# Autodesk Inventor assembly: robot
(part 2 of 2)
- Insert:483: servo frame mg996 centered_MIR_MIR:1 ↔ m2 nuts:23
## Named parameters: d57_d28 = 0 mm, d58_d29 = 0 mm, d59_d16 = 0 mm, d60_d17 = 0 deg, d61_d18 = 0 mm, d62_d19 = 0 mm, d63_d20 = 0 mm, d64_d21 = 0 mm, d65_d22 = 0 mm, d66_d23 = 0 mm, d67_d24 = 0 mm, d68_d25 = 0 mm, d69_d26 = 0 mm, d70_d27 = 0 mm, d71_d5 = 0 mm, d72_d6 = 0 mm, d73_d7 = 0 mm, d74_d8 = 0 mm, d75_d9 = 0 mm, d76_d10 = 0 mm, d77_d11 = 0 mm, d78_d12 = 0 mm, d79_d13 = 0 mm, d80_d14 = 0 mm, d81_d0 = 0 mm, d82_d1 = 0 mm, d83_d2 = 0 mm, d88_d0 = 0 mm, d89_d1 = 0 mm, d90_d2 = 0 mm, d91_d5 = 0 mm, d92_d6 = 0 mm, d93_d7 = 0 mm, d94_d8 = 0 mm, d95_d9 = 0 mm, d96_d10 = 0 mm, d97_d11 = 0 mm, d98_d12 = 0 mm, d99_d13 = 0 mm, d100_d14 = 0 mm, d101_d16 = 0 mm, d102_d17 = 0 deg, d103_d18 = 0 mm, d104_d19 = 0 mm, d105_d20 = 0 mm, d106_d21 = 0 mm, d107_d22 = 0 mm, d108_d23 = 0 mm, d109_d24 = 0 mm, d110_d25 = 0 mm, d111_d26 = 0 mm, d112_d27 = 0 mm, d113_d28 = 0 mm, d114_d29 = 0 mm, d118_d0 = 0 mm, d119_d1 = 0 mm, d120_d2 = 0 mm, d121_d5 = 0 mm, d122_d6 = 0 mm, d123_d7 = 0 mm, d124_d8 = 0 mm, d125_d9 = 0 mm, d126_d10 = 0 mm, d127_d11 = 0 mm, d128_d12 = 0 mm, d129_d13 = 0 mm, d130_d14 = 0 mm, d131_d16 = 0 mm, d132_d17 = -0.006232 deg, d133_d22 = 0 mm, d134_d23 = 0 mm, d135_d24 = 0 mm, d136_d25 = 0 mm, d146_d0 = 0 mm, d147_d1 = 0 mm, d148_d2 = 0 mm, d149_d5 = 0 mm, d150_d6 = 0 mm, d151_d7 = 0 mm, d152_d8 = 0 mm, d153_d9 = 0 mm, d154_d10 = 0 mm, d155_d11 = 0 mm, d156_d12 = 0 mm, d157_d13 = 0 mm, d158_d14 = 0 mm, d159_d16 = 0 mm, d160_d17 = 2.549165 deg, d161_d22 = 0 mm, d162_d23 = 0 mm, d163_d24 = 0 mm, d164_d25 = 0 mm, d175_d118_d0 = 0 mm, d176_d119_d1 = 0 mm, d177_d120_d2 = 0 mm, d178_d121_d5 = 0 mm, d179_d122_d6 = 0 mm, d180_d123_d7 = 0 mm, d181_d124_d8 = 0 mm, d182_d125_d9 = 0 mm, d183_d126_d10 = 0 mm, d184_d127_d11 = 0 mm, d185_d128_d12 = 0 mm, d186_d131_d16 = 0 mm, d187_d132_d17 = 0.807416 deg, d188_d133_d22 = 0 mm, d189_d134_d23 = 0 mm, d190_d135_d24 = 0 mm, d191_d136_d25 = 0 mm, d298_d175_d118_d0 = 0 mm, d299_d176_d119_d1 = 0 mm, d300_d177_d120_d2 = 0 mm, d301_d178_d121_d5 = 0 mm, d302_d179_d122_d6 = 0 mm, d303_d180_d123_d7 = 0 mm, d304_d181_d124_d8 = 0 mm, d305_d182_d125_d9 = 0 mm, d306_d183_d126_d10 = 0 mm, d307_d184_d127_d11 = 0 mm, d308_d185_d128_d12 = 0 mm, d309_d186_d131_d16 = 0 mm, d310_d187_d132_d17 = 5.394819 deg
